# Autodesk Inventor assembly: 車軸受け
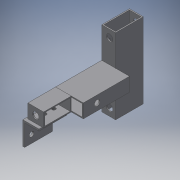
[picture p0: Inventor's stored thumbnail of the model, 180x180]
Saved by Autodesk Inventor 2018 (Build 220112000, 112)
## iProperties
Created: 2017-09-15
Part Number: 車軸受け
Material: 一般
Document SubType Name: Assembly
Designer: mura5
Author: mura5
## Documents named in this file (5)
- C:\Users\mura5\Documents\RBBR\CAD\サスペンション\車軸受け(後,左).iam
- C:\Users\mura5\Documents\RBBR\CAD\サスペンション\車軸受け1.ipt
- C:\Users\mura5\Documents\RBBR\CAD\サスペンション\車軸受け2.ipt
- C:\Users\mura5\Documents\RBBR\CAD\サスペンション\車軸受け3.ipt
- C:\Users\mura5\Documents\RBBR\CAD\サスペンション\ブレーキ固定アングル.ipt
## Components (4 placed, 4 different names)
1. 車軸受け1:1 — リジッド:2, フラッシュ:1, メイト:1, フラッシュ:2, メイト:3
2. 車軸受け3:1 — フラッシュ:1, メイト:1, フラッシュ:2
3. 車軸受け2:2 — リジッド:2, メイト:2, フラッシュ:3
4. ブレーキ固定アングル:1 — メイト:2, フラッシュ:3, メイト:3
## Relationships (7: Flush 3, Mate 3, WeldJoint 1)
- リジッド:2 [WeldJoint]: 車軸受け1:1 ↔ 車軸受け2:2
- フラッシュ:1 [Flush]: 車軸受け1:1 ↔ 車軸受け3:1
- メイト:1 [Mate]: 車軸受け1:1 ↔ 車軸受け3:1
- フラッシュ:2 [Flush] (66.75 mm): 車軸受け1:1 ↔ 車軸受け3:1
- メイト:2 [Mate]: 車軸受け2:2 ↔ ブレーキ固定アングル:1
- フラッシュ:3 [Flush] (3 mm): 車軸受け2:2 ↔ ブレーキ固定アングル:1
- メイト:3 [Mate] (7 mm): 車軸受け1:1 ↔ ブレーキ固定アングル:1
